# Autodesk Inventor assembly: Conveyor
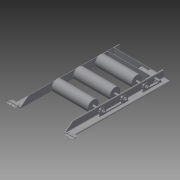
[picture p0: Inventor's stored thumbnail of the model, 180x180]
Saved by Autodesk Inventor 2015 (Build 190159000, 159)
## iProperties
Created: 2015-01-11
Part Number: Conveyor
Document SubType Name: Assembly
Designer: chapale16
Author: chapale16
## Documents named in this file (8)
- \\lhssvr02\Homedirs\Robotics Club\CAD Model 2015\Box Beam Drive Base\Conveyor.iam
- \\lhssvr02\Homedirs\Robotics Club\CAD Model 2015\Box Beam Drive Base\Axle With single sprocket.iam
- \\lhssvr02\Homedirs\Robotics Club\CAD Model 2015\Game Components\The Tote Collector-Arms\P60 Gear Box.ipt
- \\lhssvr02\Homedirs\Robotics Club\CAD Model 2015\Box Beam Drive Base\Conveyor Brace.ipt
- H:\Sprocket Large.ipt
- \\lhssvr02\Homedirs\Robotics Club\CAD Model 2015\CDR prep\Frame\2x2 quarter in angle aluminum number 2.ipt
- \\lhssvr02\Homedirs\Robotics Club\CAD Model 2015\CDR prep\Frame\2x2 quarter in angle aluminum far side.ipt
- \\lhssvr02\Homedirs\Robotics Club\CAD Model 2015\Box Beam Drive Base\door hinge for arms.iam
## Components (11 placed, 7 different names)
1. Axle With single sprocket:1 [sub-assembly] — Mate:37, Flush:6
2. P60 Gear Box:2 — Mate:18, Mate:19, Mate:20, Mate:41, Mate:42, Mate:43, Flush:8
3. Conveyor Brace:1 — Mate:18, Flush:1, Mate:34, Mate:40, Flush:9
4. Conveyor Brace:2 — Mate:19, Flush:2, Mate:33, Mate:44
5. Sprocket Large:1 — Mate:20
6. Axle With single sprocket:2 [sub-assembly] — Mate:31, Mate:32, Flush:5, Flush:6, Flush:7
7. Axle With single sprocket:3 [sub-assembly] — Mate:38, Flush:5, Flush:7, Mate:40, Flush:8
8. 2x2 quarter in angle aluminum number 2:1 — Mate:31, Mate:32, Flush:1, Flush:2, Mate:33, Mate:34, Mate:37, Mate:38, Mate:41, Mate:42, Mate:43, Flush:10, Mate:46, Mate:47, Mate:48
9. 2x2 quarter in angle aluminum far side:1 — Mate:44, Flush:9, Flush:10, Flush:11, Mate:49, Mate:50
10. door hinge for arms:1 [sub-assembly] — Flush:11, Mate:49, Mate:50
11. door hinge for arms:2 [sub-assembly] — Mate:46, Mate:47, Mate:48
## Relationships (28: Mate 19, Flush 9)
- Mate:18: P60 Gear Box:2 ↔ Conveyor Brace:1
- Mate:19: P60 Gear Box:2 ↔ Conveyor Brace:2
- Mate:20: P60 Gear Box:2 ↔ Sprocket Large:1
- Mate:31: Axle With single sprocket:2 ↔ 2x2 quarter in angle aluminum number 2:1
- Mate:32: Axle With single sprocket:2 ↔ 2x2 quarter in angle aluminum number 2:1
- Flush:1: Conveyor Brace:1 ↔ 2x2 quarter in angle aluminum number 2:1
- Flush:2: Conveyor Brace:2 ↔ 2x2 quarter in angle aluminum number 2:1
- Mate:33: Conveyor Brace:2 ↔ 2x2 quarter in angle aluminum number 2:1
- Mate:34: Conveyor Brace:1 ↔ 2x2 quarter in angle aluminum number 2:1
- Mate:37: Axle With single sprocket:1 ↔ 2x2 quarter in angle aluminum number 2:1
- Mate:38: Axle With single sprocket:3 ↔ 2x2 quarter in angle aluminum number 2:1
- Flush:5: Axle With single sprocket:2 ↔ Axle With single sprocket:3
- Flush:6: Axle With single sprocket:1 ↔ Axle With single sprocket:2
- Flush:7: Axle With single sprocket:2 ↔ Axle With single sprocket:3
- Mate:40 (57.15 mm): Conveyor Brace:1 ↔ Axle With single sprocket:3
- Mate:41: P60 Gear Box:2 ↔ 2x2 quarter in angle aluminum number 2:1
- Mate:42: P60 Gear Box:2 ↔ 2x2 quarter in angle aluminum number 2:1
- Mate:43: P60 Gear Box:2 ↔ 2x2 quarter in angle aluminum number 2:1
- Flush:8: P60 Gear Box:2 ↔ Axle With single sprocket:3
- Mate:44: Conveyor Brace:2 ↔ 2x2 quarter in angle aluminum far side:1
- Flush:9: Conveyor Brace:1 ↔ 2x2 quarter in angle aluminum far side:1
- Flush:10: 2x2 quarter in angle aluminum number 2:1 ↔ 2x2 quarter in angle aluminum far side:1
- Mate:46: 2x2 quarter in angle aluminum number 2:1 ↔ door hinge for arms:2
- Mate:47: 2x2 quarter in angle aluminum number 2:1 ↔ door hinge for arms:2
- Mate:48 (6.35 mm): 2x2 quarter in angle aluminum number 2:1 ↔ door hinge for arms:2
- Flush:11: 2x2 quarter in angle aluminum far side:1 ↔ door hinge for arms:1
- Mate:49: 2x2 quarter in angle aluminum far side:1 ↔ door hinge for arms:1
- Mate:50 (6.35 mm): 2x2 quarter in angle aluminum far side:1 ↔ door hinge for arms:1
